# Autodesk Inventor assembly: Hot End Assembly
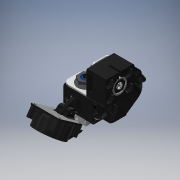
[picture p0: Inventor's stored thumbnail of the model, 180x180]
Saved by Autodesk Inventor 2019 (Build 230136000, 136)
## iProperties
Created: 2018-12-14
Part Number: Hot End Assembly
Document SubType Name: Assembly
Designer: Ax
Author: Ax
## Documents named in this file (10)
- C:\Users\Ax\Google Drive\Inventor\AX-01\Hot End Assembly.iam
- C:\Users\Ax\Google Drive\Inventor\Library\E3Dv6_1_75mm_Threaded_Heatsink .iam
- C:\Users\Ax\Google Drive\Inventor\Library\Hot_End_Fan.ipt
- C:\Users\Ax\Google Drive\Inventor\Library\Layer_Fan_Mount.ipt
- C:\Users\Ax\Google Drive\Inventor\Library\30mm Fan.ipt
- C:\Users\Ax\Google Drive\Inventor\Library\blower_fan.ipt
- C:\Users\Ax\Google Drive\Inventor\AX-01\Hot End Mount.ipt
- C:\Users\Ax\Google Drive\Inventor\Library\Nylon Nut.ipt
- C:\Users\Ax\Google Drive\Inventor\AX-01\Electromagnet Block.ipt
- C:\Users\Ax\Google Drive\Inventor\AX-01\20-15 Electromagnet.ipt
## Components (11 placed, 9 different names)
1. E3Dv6_1_75mm_Threaded_Heatsink :1 [sub-assembly] — Mate:1, Mate:2, Flush:1, Rigid:1, Rigid:4
2. Hot_End_Fan:1 — Rigid:1, Rigid:2, Rigid:3, Mate:3, Mate:4, Mate:5
3. Layer_Fan_Mount:1 — Rigid:2, Mate:6, Mate:7, Mate:8
4. Layer_Fan_Mount:2 — Rigid:3, Mate:9, Mate:10, Mate:11
5. 30mm Fan:1 — Mate:3, Mate:4, Mate:5
6. blower_fan:1 — Mate:6, Mate:7, Mate:8
7. blower_fan:2 — Mate:9, Mate:10, Mate:11
8. Hot End Mount:1 — Rigid:4, Rigid:5, Mate:12, Mate:13, Mate:14
9. Nylon Nut:1 — Rigid:5
10. Electromagnet Block:1 — Mate:12, Mate:13, Mate:14, Mate:15, Mate:16
11. 20-15 Electromagnet:1 — Mate:15, Mate:16
## Relationships (22: Mate 16, WeldJoint 5, Flush 1)
- Mate:1: E3Dv6_1_75mm_Threaded_Heatsink :1
- Mate:2: E3Dv6_1_75mm_Threaded_Heatsink :1
- Flush:1: E3Dv6_1_75mm_Threaded_Heatsink :1
- Rigid:1 [WeldJoint] (2 mm): E3Dv6_1_75mm_Threaded_Heatsink :1 ↔ Hot_End_Fan:1
- Rigid:2 [WeldJoint]: Hot_End_Fan:1 ↔ Layer_Fan_Mount:1
- Rigid:3 [WeldJoint]: Hot_End_Fan:1 ↔ Layer_Fan_Mount:2
- Mate:3: Hot_End_Fan:1 ↔ 30mm Fan:1
- Mate:4: Hot_End_Fan:1 ↔ 30mm Fan:1
- Mate:5: Hot_End_Fan:1 ↔ 30mm Fan:1
- Mate:6: Layer_Fan_Mount:1 ↔ blower_fan:1
- Mate:7: Layer_Fan_Mount:1 ↔ blower_fan:1
- Mate:8: Layer_Fan_Mount:1 ↔ blower_fan:1
- Mate:9: Layer_Fan_Mount:2 ↔ blower_fan:2
- Mate:10: Layer_Fan_Mount:2 ↔ blower_fan:2
- Mate:11: Layer_Fan_Mount:2 ↔ blower_fan:2
- Rigid:4 [WeldJoint]: E3Dv6_1_75mm_Threaded_Heatsink :1 ↔ Hot End Mount:1
- Rigid:5 [WeldJoint]: Hot End Mount:1 ↔ Nylon Nut:1
- Mate:12: Hot End Mount:1 ↔ Electromagnet Block:1
- Mate:13: Hot End Mount:1 ↔ Electromagnet Block:1
- Mate:14: Hot End Mount:1 ↔ Electromagnet Block:1
- Mate:15: Electromagnet Block:1 ↔ 20-15 Electromagnet:1
- Mate:16: Electromagnet Block:1 ↔ 20-15 Electromagnet:1
